# Autodesk Inventor assembly: mainflap_center
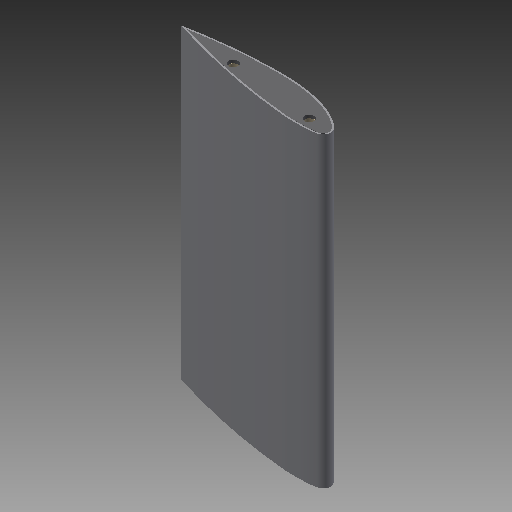
[picture p0: Inventor's stored thumbnail of the model, 512x512]
Saved by Autodesk Inventor 2018 (Build 220112000, 112)
## iProperties
Created: 2018-03-05
Part Number: mainflap_center
Material: 一般
Document SubType Name: Assembly
Designer: ku_sk
Author: ku_sk
## Documents named in this file (4)
- D:\Users\ku_sk\Documents\Inventor\Aero\KS-15\Fr.wing\parts\mainflap_center\mainflap_center.iam
- D:\Users\ku_sk\Documents\Inventor\Aero\KS-15\Fr.wing\parts\mainflap_center\plate_mc.ipt
- D:\Users\ku_sk\Documents\Inventor\Aero\KS-15\Fr.wing\parts\mainflap_center\uretan_mc.ipt
- D:\Users\ku_sk\Documents\Inventor\Aero\KS-15\Fr.wing\parts\mainflap_center\GFRP_mc.ipt
## Components (18 placed, 3 different names)
1. plate_mc:1 — メイト:3, メイト:4, フラッシュ:10, メイト:28, メイト:29, メイト:30, メイト:31, メイト:32, メイト:36, メイト:37, メイト:38, メイト:39, メイト:40, メイト:41, メイト:42
2. plate_mc:2 — メイト:2, メイト:3, メイト:4, フラッシュ:2, メイト:5, メイト:6, メイト:20, フラッシュ:13
3. plate_mc:3 — フラッシュ:2, フラッシュ:3, メイト:5, メイト:6, メイト:7, メイト:8, メイト:21, メイト:43
4. plate_mc:4 — フラッシュ:3, フラッシュ:4, メイト:7, メイト:8, メイト:9, メイト:10, メイト:22, メイト:33, メイト:34, メイト:35
5. plate_mc:5 — フラッシュ:4, フラッシュ:5, メイト:9, メイト:10, メイト:11, メイト:12, メイト:23
6. plate_mc:6 — フラッシュ:5, メイト:11, メイト:12, フラッシュ:11, フラッシュ:12, メイト:24
7. plate_mc:8 — フラッシュ:8, メイト:17, メイト:18, フラッシュ:11, メイト:25
8. plate_mc:9 — フラッシュ:8, フラッシュ:9, メイト:17, メイト:18, メイト:19, メイト:26
9. plate_mc:10 — フラッシュ:9, メイト:19, フラッシュ:10, メイト:27
10. uretan_mc:1 — メイト:20, メイト:34, メイト:42, メイト:45
11. uretan_mc:2 — メイト:21, メイト:33, メイト:43, メイト:44
12. uretan_mc:3 — メイト:22, メイト:35, メイト:41
13. uretan_mc:4 — メイト:23, メイト:32, メイト:40
14. uretan_mc:5 — メイト:24, メイト:31, メイト:39
15. uretan_mc:6 — メイト:25, メイト:30, メイト:38
16. uretan_mc:7 — メイト:26, メイト:29, メイト:37
17. uretan_mc:8 — メイト:27, メイト:28, メイト:36
18. GFRP_mc:1 — メイト:44, メイト:45, フラッシュ:13
## Relationships (50: Mate 40, Flush 10)
- メイト:2 [Mate]: plate_mc:2
- メイト:3 [Mate]: plate_mc:1 ↔ plate_mc:2
- メイト:4 [Mate]: plate_mc:1 ↔ plate_mc:2
- フラッシュ:2 [Flush] (48.75 mm): plate_mc:2 ↔ plate_mc:3
- フラッシュ:3 [Flush] (-48.75 mm): plate_mc:3 ↔ plate_mc:4
- フラッシュ:4 [Flush] (48.75 mm): plate_mc:4 ↔ plate_mc:5
- フラッシュ:5 [Flush] (-48.75 mm): plate_mc:5 ↔ plate_mc:6
- メイト:5 [Mate]: plate_mc:2 ↔ plate_mc:3
- メイト:6 [Mate]: plate_mc:2 ↔ plate_mc:3
- メイト:7 [Mate]: plate_mc:3 ↔ plate_mc:4
- メイト:8 [Mate]: plate_mc:3 ↔ plate_mc:4
- メイト:9 [Mate]: plate_mc:4 ↔ plate_mc:5
- メイト:10 [Mate]: plate_mc:4 ↔ plate_mc:5
- メイト:11 [Mate]: plate_mc:5 ↔ plate_mc:6
- メイト:12 [Mate]: plate_mc:5 ↔ plate_mc:6
- フラッシュ:8 [Flush] (-48.75 mm): plate_mc:8 ↔ plate_mc:9
- フラッシュ:9 [Flush] (-48.75 mm): plate_mc:9 ↔ plate_mc:10
- メイト:17 [Mate]: plate_mc:8 ↔ plate_mc:9
- メイト:18 [Mate]: plate_mc:8 ↔ plate_mc:9
- メイト:19 [Mate]: plate_mc:9 ↔ plate_mc:10
- フラッシュ:10 [Flush] (-48.75 mm): plate_mc:1 ↔ plate_mc:10
- フラッシュ:11 [Flush] (48.75 mm): plate_mc:6 ↔ plate_mc:8
- フラッシュ:12 [Flush] (-2 mm): plate_mc:6
- メイト:20 [Mate]: plate_mc:2 ↔ uretan_mc:1
- メイト:21 [Mate]: plate_mc:3 ↔ uretan_mc:2
- メイト:22 [Mate]: plate_mc:4 ↔ uretan_mc:3
- メイト:23 [Mate]: plate_mc:5 ↔ uretan_mc:4
- メイト:24 [Mate]: plate_mc:6 ↔ uretan_mc:5
- メイト:25 [Mate]: plate_mc:8 ↔ uretan_mc:6
- メイト:26 [Mate]: plate_mc:9 ↔ uretan_mc:7
- メイト:27 [Mate]: plate_mc:10 ↔ uretan_mc:8
- メイト:28 [Mate]: plate_mc:1 ↔ uretan_mc:8
- メイト:29 [Mate]: plate_mc:1 ↔ uretan_mc:7
- メイト:30 [Mate]: plate_mc:1 ↔ uretan_mc:6
- メイト:31 [Mate]: plate_mc:1 ↔ uretan_mc:5
- メイト:32 [Mate]: plate_mc:1 ↔ uretan_mc:4
- メイト:33 [Mate]: plate_mc:4 ↔ uretan_mc:2
- メイト:34 [Mate]: plate_mc:4 ↔ uretan_mc:1
- メイト:35 [Mate]: plate_mc:4 ↔ uretan_mc:3
- メイト:36 [Mate]: plate_mc:1 ↔ uretan_mc:8
- メイト:37 [Mate]: plate_mc:1 ↔ uretan_mc:7
- メイト:38 [Mate]: plate_mc:1 ↔ uretan_mc:6
- メイト:39 [Mate]: plate_mc:1 ↔ uretan_mc:5
- メイト:40 [Mate]: plate_mc:1 ↔ uretan_mc:4
- メイト:41 [Mate]: plate_mc:1 ↔ uretan_mc:3
- メイト:42 [Mate]: plate_mc:1 ↔ uretan_mc:1
- メイト:43 [Mate]: plate_mc:3 ↔ uretan_mc:2
- メイト:44 [Mate]: uretan_mc:2 ↔ GFRP_mc:1
- メイト:45 [Mate]: uretan_mc:1 ↔ GFRP_mc:1
- フラッシュ:13 [Flush]: plate_mc:2 ↔ GFRP_mc:1
